# Autodesk Inventor assembly: Montaje Motor - V2
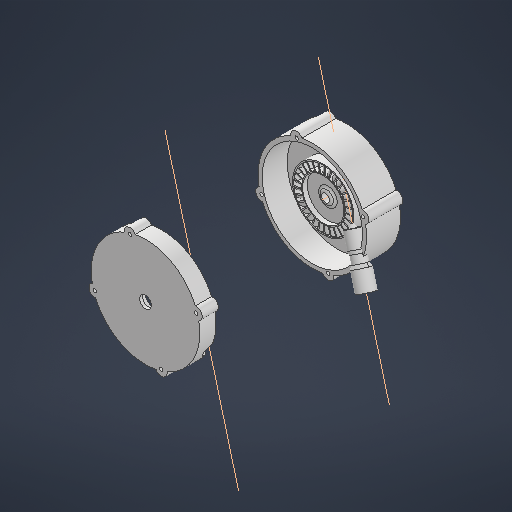
[picture p0: Inventor's stored thumbnail of the model, 512x512]
Saved by Autodesk Inventor 2025.3 (Build 293356030, 356C)
## iProperties
Created: 2025-09-18
Part Number: Montaje Motor - V2
Document SubType Name: Assembly
Designer: yo
Author: yo
## Documents named in this file (6)
- C:\Users\yo\Documents\Andes\9no Semestre\Proyecto Intermedio\Proyecto\Huron-Hudson\Versions\V2\Montaje Motor - V2.iam
- C:\Users\yo\Documents\Andes\9no Semestre\Proyecto Intermedio\Proyecto\Huron-Hudson\Versions\V2\Case Part 1 - V2.ipt
- C:\Users\yo\Documents\Andes\9no Semestre\Proyecto Intermedio\Proyecto\Huron-Hudson\Versions\V2\Case Part 2 - V2.ipt
- C:\Users\yo\Documents\Andes\9no Semestre\Proyecto Intermedio\Proyecto\Huron-Hudson\Versions\V2\Pelton - V2.ipt
- C:\Users\yo\Documents\Andes\9no Semestre\Proyecto Intermedio\Proyecto\Huron-Hudson\Versions\V2\Nozzle.ipt
- C:\Users\yo\Documents\Andes\9no Semestre\Proyecto Intermedio\Proyecto\Huron-Hudson\Versions\V2\Reductor.ipt
## Components (5 placed, 5 different names)
1. Case Part 1 - V2:1 — Mate:1, Mate:2, Mate:3, Mate:4, Mate:5, Mate:6, Mate:7, Mate:8
2. Case Part 2 - V2:1 — Mate:3, Mate:4
3. Pelton - V2:1 — Mate:5, Mate:6
4. Nozzle:1 — Mate:7
5. Reductor:1 — Mate:8
## Relationships (8: Mate 8)
- Mate:1: Case Part 1 - V2:1
- Mate:2: Case Part 1 - V2:1
- Mate:3: Case Part 1 - V2:1 ↔ Case Part 2 - V2:1
- Mate:4: Case Part 1 - V2:1 ↔ Case Part 2 - V2:1
- Mate:5: Case Part 1 - V2:1 ↔ Pelton - V2:1
- Mate:6 (2 mm): Case Part 1 - V2:1 ↔ Pelton - V2:1
- Mate:7: Case Part 1 - V2:1 ↔ Nozzle:1
- Mate:8: Case Part 1 - V2:1 ↔ Reductor:1
